# Autodesk Inventor assembly: Assembly2 стойка
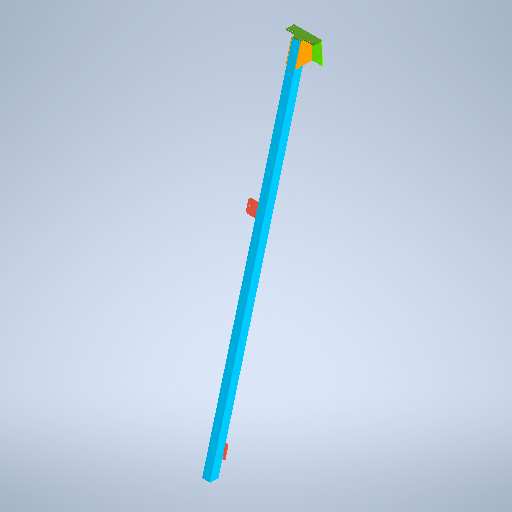
[picture p0: Inventor's stored thumbnail of the model, 512x512]
Saved by Autodesk Inventor 2025 (Build 290162010, 162A)
## iProperties
Created: 2024-06-18
Part Number: Assembly2 стойка
Document SubType Name: Assembly
Designer: admin
Author: admin
## Documents named in this file (7)
- C:\Users\admin\YandexDisk-badmisterfox\домашниий пк\Inventor\Workshop\оборудование\Кран козловой 2\Assembly2 стойка.iam
- C:\Users\admin\YandexDisk-badmisterfox\домашниий пк\Inventor\Workshop\оборудование\Кран козловой 2\полка под швеллер.ipt
- C:\Users\admin\YandexDisk-badmisterfox\домашниий пк\Inventor\Workshop\оборудование\Кран козловой 2\стойка 1 100x100x4 - 5000.ipt
- C:\Users\admin\YandexDisk-badmisterfox\домашниий пк\Inventor\Workshop\оборудование\Кран козловой 2\держатель полки 1.ipt
- C:\Users\admin\YandexDisk-badmisterfox\домашниий пк\Inventor\Workshop\оборудование\Кран козловой 2\Ухо на стойку.ipt
- C:\Users\admin\YandexDisk-badmisterfox\домашниий пк\Inventor\Workshop\оборудование\Кран козловой 2\Ухо на швеллер пямое_CPY.ipt
- C:\Users\admin\YandexDisk-badmisterfox\домашниий пк\Inventor\Workshop\оборудование\Кран козловой 2\Ухо на стойку_CPY.ipt
## Components (7 placed, 6 different names)
1. полка под швеллер:1
2. стойка 1 100x100x4 - 5000:1
3. держатель полки 1:1
4. Ухо на стойку:1
5. держатель полки 1:2
6. Ухо на швеллер пямое_CPY:1
7. Ухо на стойку_CPY:1
## Relationships (15: Mate 9, Flush 5, WeldJoint 1)
- [Mate]: стойка 1 100x100x4 - 5000:1 ↔ держатель полки 1:1
- [Mate]: стойка 1 100x100x4 - 5000:1 ↔ держатель полки 1:2
- [Flush]: стойка 1 100x100x4 - 5000:1 ↔ держатель полки 1:2
- [Flush]: стойка 1 100x100x4 - 5000:1 ↔ держатель полки 1:1
- [Flush]: стойка 1 100x100x4 - 5000:1 ↔ держатель полки 1:1
- [Flush]: стойка 1 100x100x4 - 5000:1 ↔ держатель полки 1:2
- [WeldJoint]: полка под швеллер:1 ↔ Ухо на швеллер пямое_CPY:1
- [Flush]: стойка 1 100x100x4 - 5000:1 ↔ Ухо на швеллер пямое_CPY:1
- [Mate]: стойка 1 100x100x4 - 5000:1 ↔ Ухо на швеллер пямое_CPY:1
- [Mate]: стойка 1 100x100x4 - 5000:1 ↔ Ухо на стойку:1
- [Mate]: стойка 1 100x100x4 - 5000:1 ↔ Ухо на стойку:1
- [Mate]: полка под швеллер:1 ↔ держатель полки 1:2
- [Mate] (-200 mm): стойка 1 100x100x4 - 5000:1 ↔ Ухо на стойку:1
- [Mate]: стойка 1 100x100x4 - 5000:1 ↔ Ухо на стойку_CPY:1
- [Mate]: стойка 1 100x100x4 - 5000:1 ↔ Ухо на стойку_CPY:1
